# Autodesk Inventor assembly: frame
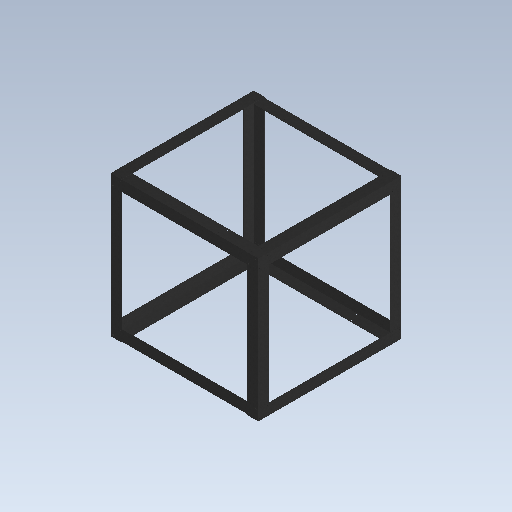
[picture p0: Inventor's stored thumbnail of the model, 512x512]
Saved by Autodesk Inventor 2020.4 (Build 244396000, 396)
## iProperties
Created: 2021-02-28
Part Number: frame
Document SubType Name: Assembly
Designer: AOB
Mass: 5666.96 g
Surface Area: 9341.55 cm^2
Volume: 721.905 cm^3
Density: 7.85 g/cm^3
Author: AOB
## Documents named in this file (5)
- C:\Users\marti\Documents\Inventor\ProjectBoron\Boron Ultima\frame.iam
- C:\Users\marti\Documents\Inventor\ProjectBoron\Boron Ultima\angleline-500.ipt
- C:\Users\marti\Documents\Inventor\ProjectBoron\Boron Ultima\angleline-400.ipt
- C:\Users\marti\Documents\Inventor\ProjectBoron\Boron Ultima\angleline-cross-400.ipt
- C:\Users\marti\Documents\Inventor\ProjectBoron\Boron Ultima\frame-back.iam
## Components (9 placed, 4 different names)
1. angleline-500:1 — Mate:4, Mate:5, Mate:12, Mate:13, Mate:14, Mate:15
2. angleline-500:2 — Mate:1, Mate:2, Mate:6, Mate:7, Mate:8, Mate:9, Mate:10, Mate:11
3. angleline-430:1 — Mate:1, Mate:2, Mate:4, Mate:5
4. angleline-430:2 — Mate:6, Mate:7
5. angleline-cross-400:1 — Mate:8, Mate:9, Mate:16, Mate:17
6. angleline-cross-400:2 — Mate:12, Mate:13
7. angleline-cross-400:4 — Mate:14, Mate:15, Mate:18, Mate:19
8. angleline-cross-400:3 — Mate:10, Mate:11
9. frame-back:1 [sub-assembly] — Mate:16, Mate:17, Mate:18, Mate:19
## Relationships (18: Mate 18)
- Mate:1: angleline-500:2 ↔ angleline-430:1
- Mate:2: angleline-500:2 ↔ angleline-430:1
- Mate:4: angleline-500:1 ↔ angleline-430:1
- Mate:5: angleline-500:1 ↔ angleline-430:1
- Mate:6: angleline-500:2 ↔ angleline-430:2
- Mate:7: angleline-500:2 ↔ angleline-430:2
- Mate:8: angleline-500:2 ↔ angleline-cross-400:1
- Mate:9: angleline-500:2 ↔ angleline-cross-400:1
- Mate:10: angleline-500:2 ↔ angleline-cross-400:3
- Mate:11: angleline-500:2 ↔ angleline-cross-400:3
- Mate:12: angleline-500:1 ↔ angleline-cross-400:2
- Mate:13: angleline-500:1 ↔ angleline-cross-400:2
- Mate:14: angleline-500:1 ↔ angleline-cross-400:4
- Mate:15: angleline-500:1 ↔ angleline-cross-400:4
- Mate:16: angleline-cross-400:1 ↔ frame-back:1
- Mate:17: angleline-cross-400:1 ↔ frame-back:1
- Mate:18: angleline-cross-400:4 ↔ frame-back:1
- Mate:19: angleline-cross-400:4 ↔ frame-back:1
